# Autodesk Inventor assembly: Spinn5_Enclosure
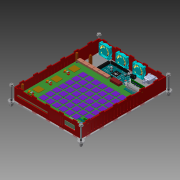
[picture p0: Inventor's stored thumbnail of the model, 180x180]
Saved by Autodesk Inventor 2015 SP1 (Build 190203100, 203)
## iProperties
Created: 2014-08-07
Part Number: Spinn5_Enclosure
Document SubType Name: Assembly
Designer: Patrick Camilleri
Author: Patrick Camilleri
## Documents named in this file (15)
- C:\Users\Patrick\EDA\CAD\Spin4 Enclosure\Spinn4_Enclosure.iam
- C:\Users\Patrick\EDA\CAD\Spin4 Enclosure\BasePlate.ipt
- C:\Users\Patrick\EDA\CAD\Spin4 Enclosure\SidePanel.ipt
- C:\Users\Patrick\EDA\CAD\Spin4 Enclosure\SidePanelFans2.iam
- C:\Users\Patrick\EDA\CAD\Spin4 Enclosure\BoltAssembly.iam
- C:\Users\Patrick\EDA\CAD\Spin4 Enclosure\Stopper.ipt
- C:\Users\Patrick\EDA\CAD\Spin5 PowerPcb\Imported Components\Spinn5Power\Spinn5Power.iam
- C:\Users\Patrick\EDA\CAD\Spin4 Enclosure\SidePanel_v2_left.iam
- C:\Users\Patrick\EDA\CAD\Spin4 Enclosure\SidePanel_v2_right.iam
- C:\Users\Patrick\EDA\CAD\Spin4 Enclosure\TopPlate2.ipt
- C:\Users\Patrick\EDA\CAD\Spin4 Board\spin4v23.brd1.iam
- C:\Users\Patrick\EDA\CAD\ARDUINO DUE\ARDUINO DUE.iam
- C:\Users\Patrick\EDA\PCBs\Spin3\Spacer M3x5mm.ipt
- C:\Users\Patrick\EDA\CAD\Spin4 Enclosure\Imported Components\M3x0_5xL Phillips Panhead Screw15mm\M3x0_5xL Phillips Panhead Screw15mm.ipt
- C:\Users\Patrick\EDA\CAD\Spin4 Enclosure\Imported Components\HEX PLAIN and NYLOC METRIC\HEX PLAIN and NYLOC METRIC.ipt
## Components (26 placed, 14 different names)
1. BasePlate:1 — Rigid:19, Rigid:29, Rigid:32, Rigid:33, Rigid:34, Mate:1, Mate:2, Mate:3, Mate:4, Mate:5, Mate:6, Mate:7, Mate:8, Mate:9, Mate:16, Mate:17, Mate:18, Mate:19, Mate:20, Mate:21, Mate:22, Mate:23, Mate:24, Mate:25, Mate:31, Mate:32, Mate:33, Mate:34
2. SidePanel:1 — Rigid:32
3. BoltAssembly:1 [sub-assembly] — Mate:4, Mate:5
4. BoltAssembly:2 [sub-assembly] — Mate:8, Mate:9
5. BoltAssembly:3 [sub-assembly] — Mate:6, Mate:7
6. BoltAssembly:4 [sub-assembly] — Mate:1, Mate:2, Mate:3
7. Stopper:1 — Rigid:19, Mate:12
8. SidePanelFans2:1 [sub-assembly] — Rigid:34
9. Spinn5Power:1 [sub-assembly] — Mate:13, Mate:14, Mate:15
10. SidePanel_v2_left:1 [sub-assembly] — Rigid:29, Mate:10, Mate:11
11. SidePanel_v2_right:1 [sub-assembly] — Rigid:33
12. TopPlate2:1
13. spin4v23.brd:1 [sub-assembly] — Mate:10, Mate:11, Mate:12, Mate:13, Mate:14, Mate:15
14. ARDUINO DUE:1 [sub-assembly] — Mate:16, Mate:17, Mate:26, Mate:39, Mate:40, Mate:41, Mate:42
15. Spacer M3x5mm:1 — Mate:18, Mate:22, Mate:26, Mate:27
16. Spacer M3x5mm:2 — Mate:19, Mate:23, Mate:28
17. Spacer M3x5mm:3 — Mate:21, Mate:25, Mate:30
18. Spacer M3x5mm:4 — Mate:20, Mate:24, Mate:29
19. M3x0_5xL Phillips Panhead Screw15mm:1 — Mate:27, Mate:32, Mate:37
20. M3x0_5xL Phillips Panhead Screw15mm:2 — Mate:28, Mate:31, Mate:35
21. M3x0_5xL Phillips Panhead Screw15mm:3 — Mate:29, Mate:33, Mate:38
22. M3x0_5xL Phillips Panhead Screw15mm:4 — Mate:30, Mate:34, Mate:36
23. HEX PLAIN and NYLOC METRIC:1 — Mate:35, Mate:39
24. HEX PLAIN and NYLOC METRIC:2 — Mate:36, Mate:41
25. HEX PLAIN and NYLOC METRIC:3 — Mate:37, Mate:40
26. HEX PLAIN and NYLOC METRIC:4 — Mate:38, Mate:42
## Relationships (47: Mate 42, WeldJoint 5)
- Rigid:19 [WeldJoint]: BasePlate:1 ↔ Stopper:1
- Rigid:29 [WeldJoint]: BasePlate:1 ↔ SidePanel_v2_left:1
- Rigid:32 [WeldJoint]: BasePlate:1 ↔ SidePanel:1
- Rigid:33 [WeldJoint]: BasePlate:1 ↔ SidePanel_v2_right:1
- Rigid:34 [WeldJoint]: BasePlate:1 ↔ SidePanelFans2:1
- Mate:1: BasePlate:1 ↔ BoltAssembly:4
- Mate:2: BasePlate:1 ↔ BoltAssembly:4
- Mate:3: BasePlate:1 ↔ BoltAssembly:4
- Mate:4: BasePlate:1 ↔ BoltAssembly:1
- Mate:5: BasePlate:1 ↔ BoltAssembly:1
- Mate:6: BasePlate:1 ↔ BoltAssembly:3
- Mate:7: BasePlate:1 ↔ BoltAssembly:3
- Mate:8: BasePlate:1 ↔ BoltAssembly:2
- Mate:9: BasePlate:1 ↔ BoltAssembly:2
- Mate:10: SidePanel_v2_left:1 ↔ spin4v23.brd:1
- Mate:11: SidePanel_v2_left:1 ↔ spin4v23.brd:1
- Mate:12: Stopper:1 ↔ spin4v23.brd:1
- Mate:13: Spinn5Power:1 ↔ spin4v23.brd:1
- Mate:14: Spinn5Power:1 ↔ spin4v23.brd:1
- Mate:15: Spinn5Power:1 ↔ spin4v23.brd:1
- Mate:16: BasePlate:1 ↔ ARDUINO DUE:1
- Mate:17: BasePlate:1 ↔ ARDUINO DUE:1
- Mate:18: BasePlate:1 ↔ Spacer M3x5mm:1
- Mate:19: BasePlate:1 ↔ Spacer M3x5mm:2
- Mate:20: BasePlate:1 ↔ Spacer M3x5mm:4
- Mate:21: BasePlate:1 ↔ Spacer M3x5mm:3
- Mate:22: BasePlate:1 ↔ Spacer M3x5mm:1
- Mate:23: BasePlate:1 ↔ Spacer M3x5mm:2
- Mate:24: BasePlate:1 ↔ Spacer M3x5mm:4
- Mate:25: BasePlate:1 ↔ Spacer M3x5mm:3
- Mate:26: ARDUINO DUE:1 ↔ Spacer M3x5mm:1
- Mate:27: Spacer M3x5mm:1 ↔ M3x0_5xL Phillips Panhead Screw15mm:1
- Mate:28: Spacer M3x5mm:2 ↔ M3x0_5xL Phillips Panhead Screw15mm:2
- Mate:29: Spacer M3x5mm:4 ↔ M3x0_5xL Phillips Panhead Screw15mm:3
- Mate:30: Spacer M3x5mm:3 ↔ M3x0_5xL Phillips Panhead Screw15mm:4
- Mate:31: BasePlate:1 ↔ M3x0_5xL Phillips Panhead Screw15mm:2
- Mate:32: BasePlate:1 ↔ M3x0_5xL Phillips Panhead Screw15mm:1
- Mate:33: BasePlate:1 ↔ M3x0_5xL Phillips Panhead Screw15mm:3
- Mate:34: BasePlate:1 ↔ M3x0_5xL Phillips Panhead Screw15mm:4
- Mate:35: M3x0_5xL Phillips Panhead Screw15mm:2 ↔ HEX PLAIN and NYLOC METRIC:1
- Mate:36: M3x0_5xL Phillips Panhead Screw15mm:4 ↔ HEX PLAIN and NYLOC METRIC:2
- Mate:37: M3x0_5xL Phillips Panhead Screw15mm:1 ↔ HEX PLAIN and NYLOC METRIC:3
- Mate:38: M3x0_5xL Phillips Panhead Screw15mm:3 ↔ HEX PLAIN and NYLOC METRIC:4
- Mate:39: ARDUINO DUE:1 ↔ HEX PLAIN and NYLOC METRIC:1
- Mate:40: ARDUINO DUE:1 ↔ HEX PLAIN and NYLOC METRIC:3
- Mate:41: ARDUINO DUE:1 ↔ HEX PLAIN and NYLOC METRIC:2
- Mate:42: ARDUINO DUE:1 ↔ HEX PLAIN and NYLOC METRIC:4
